# Autodesk Inventor assembly: 足首_独立ピッチ_1
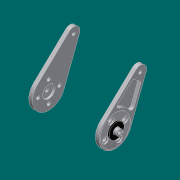
[picture p0: Inventor's stored thumbnail of the model, 180x180]
Saved by Autodesk Inventor 2016 (Build 200138000, 138)
## iProperties
Created: 2016-05-04
Part Number: 足首_独立ピッチ_1
Document SubType Name: Assembly
Designer: hiroaki
Mass: 12.4515 g
Surface Area: 78.9605 cm^2
Volume: 4.53639 cm^3
Density: 2.74481 g/cm^3
Author: hiroaki
## Documents named in this file (4)
- C:\Users\hiro\Documents\kenkyuu\二足\二足ver6.0\下半身\足首\足首_独立ピッチ_1.iam
- C:\Users\hiro\Documents\kenkyuu\二足\二足ver6.0\下半身\足首\足首_独立ピッチ_1_1.ipt
- C:\Users\hiro\Documents\kenkyuu\二足\二足ver6.0\下半身\足首\足首_独立ピッチ_1_2.ipt
- C:\Users\hiro\Documents\kenkyuu\二足\二足ver6.0\既製品\CC-0512-10B.ipt
## Components (6 placed, 3 different names)
1. 足首_独立ピッチ_1_1:1 — メイト:2, メイト:5, メイト:6, 挿入:7, 挿入:8, 挿入:9, 挿入:10
2. 足首_独立ピッチ_1_2:1 — 挿入:6, メイト:7, 挿入:7, 挿入:8, 挿入:9, 挿入:10, メイト:8
3. 足首_独立ピッチ_1_1:2 — 挿入:3, 挿入:4, メイト:2, メイト:6, 角度:1
4. 足首_独立ピッチ_1_2:2 — 挿入:3, 挿入:4, 挿入:5, メイト:7
5. CC-0512-10B:1 — 挿入:6
6. CC-0512-10B:2 — 挿入:5
## Relationships (14: Insert 8, Mate 5, Angle 1)
- 挿入:3 [Insert]: 足首_独立ピッチ_1_1:2 ↔ 足首_独立ピッチ_1_2:2
- 挿入:4 [Insert]: 足首_独立ピッチ_1_1:2 ↔ 足首_独立ピッチ_1_2:2
- メイト:2 [Mate] (50.3 mm): 足首_独立ピッチ_1_1:1 ↔ 足首_独立ピッチ_1_1:2
- メイト:5 [Mate] (25.15 mm): 足首_独立ピッチ_1_1:1
- 挿入:5 [Insert]: 足首_独立ピッチ_1_2:2 ↔ CC-0512-10B:2
- 挿入:6 [Insert]: 足首_独立ピッチ_1_2:1 ↔ CC-0512-10B:1
- メイト:6 [Mate]: 足首_独立ピッチ_1_1:1 ↔ 足首_独立ピッチ_1_1:2
- メイト:7 [Mate]: 足首_独立ピッチ_1_2:1 ↔ 足首_独立ピッチ_1_2:2
- 挿入:7 [Insert]: 足首_独立ピッチ_1_1:1 ↔ 足首_独立ピッチ_1_2:1
- 挿入:8 [Insert]: 足首_独立ピッチ_1_1:1 ↔ 足首_独立ピッチ_1_2:1
- 挿入:9 [Insert]: 足首_独立ピッチ_1_1:1 ↔ 足首_独立ピッチ_1_2:1
- 挿入:10 [Insert]: 足首_独立ピッチ_1_1:1 ↔ 足首_独立ピッチ_1_2:1
- メイト:8 [Mate]: 足首_独立ピッチ_1_2:1
- 角度:1 [Angle] (0 deg): 足首_独立ピッチ_1_1:2
